# Autodesk Inventor assembly: 19182 DSNU-8-100-P-A---(0)
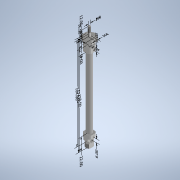
[picture p0: Inventor's stored thumbnail of the model, 180x180]
Saved by Autodesk Inventor 2021 (Build 250183000, 183)
## iProperties
Category: PARTsolutions
Company: FESTO
Created: 2026-04-16
Part Number: 19182 DSNU-8-100-P-A---(0)
Catalog Web Link: www.3dfindit.com
Description: DSNU-round cylinder
Vendor: FESTO
Document SubType Name: Assembly
Designer: psAdmin
Manufacturer: FESTO
Mass: 58.6 g
Surface Area: 124.069 cm^2
Volume: 11.6186 cm^3
Density: 5.04364 g/cm^3
Title: 19182 DSNU-8-100-P-A
Author: Cadenas PARTsolutions
Comments: round cylinder
PSOL_IDENT_0: {ATYP=ASSISTANT},{DATA=script=$CADENAS_DATA/23d-libs/festo/webfesto.vbb&M_FAMILY=DSNU&M_GROUP=01&M_P
PSOL_IDENT_1: ARTNO=19182&IDCODE1=DSNU-8-100-P-A&IDCODE2=&customer_number_cns=&MATES=1&LOD=HI&LOCKERP=0&SINGLEPART=
PSOL_IDENT_2: 1}
NB: 19182 DSNU-8-100-P-A---(0)
NN: DSNU
NT: round cylinder
NBSYN: $NB1.---($HUBST.)
LINA: 19182 DSNU-8-100-P-A
CATALOG: Festo
OFFICIAL_STANDARD_NUMBERS: ISO 6432
TNR: 19182
TYP: DSNU-8
KDM: 8
HUB: 100
HUBST: 0
DA: P
PE: A
KS: -
A1: 15
A2: 50
A3: 4
A4: 29
AB: 12
AM: 12
B: 12
BB: 3
BE: M12x1,25
BS: 3.4
B1: 24
B2: 0
B3: 0
B4: 0
B5: 14
B6: 6
B7: 0
CD: 4
D: 15
D1: 12
D2: 4
D3: 9.3
D4: 0
D5: 10.5
D6: 0
D7: 0
EE: M5
EW: 8
F: 18
FF: M3
F1: 0
H: 16
H1: 0
KK: M4
K1: -
K2: 0
KV: 19
KW: 6
KV2: 0
KW2: 0
L: 6
LH: 5
LK: 7.6
L1: 174
L2: 146
L3: 6
L4: 12
L5: 10
L6: 28
L7: 16
L8: 10
L9: 16
L13: 78
ST: 3.4
SW: 0
T: 0
WH: 16
X: 0
XC: 164
CNSMASSEXACT: 0.0586
GTIN: 4052568066949
REACH: Yes
REACHSVHC: No
REACHHAZSUBS: -
REACHSCIP: -
REACHVALDATE: -
SUPPLIER: FESTO
ARTICLENO: 19182 DSNU-8-100-P-A---(0)
BOMINFO: 19182 DSNU-8-100-P-A
CREATOR: CADENAS GmbH
## Documents named in this file (4)
- e:\temp\worker_COMMON_20\temp\tmp_2484_30_KxpFe\format_0\19182 DSNU-8-100-P-A---(0).iam
- e:\temp\worker_COMMON_20\temp\tmp_2484_30_KxpFe\format_0\19182 DSNU-8-100-P---(A----0-ZR).ipt
- e:\temp\worker_COMMON_20\temp\tmp_2484_30_KxpFe\format_0\DIN-439-B - M12x1_25(F).ipt
- e:\temp\worker_COMMON_20\temp\tmp_2484_30_KxpFe\format_0\19182 DSNU-8-100-P---(A---00--0-KS).ipt
## Components (3 placed, 3 different names)
1. 19182 DSNU-8-100-P---(A----0-ZR):1 — NUT_XY@1 <-> 2CYL_XY@2, NUT_Z@1 <-> 2CYL_Z@2, NUT_YZ@1 <-> 2CYL_YZ@2, ZR_XY@1 <-> KS_XY@3, ZR_Z@1 <-> KS_Z@3, ZR_YZ@1 <-> KS_YZ@3
2. DIN-439-B - M12x1_25(F):1 — NUT_XY@1 <-> 2CYL_XY@2, NUT_Z@1 <-> 2CYL_Z@2, NUT_YZ@1 <-> 2CYL_YZ@2
3. 19182 DSNU-8-100-P---(A---00--0-KS):1 — ZR_XY@1 <-> KS_XY@3, ZR_Z@1 <-> KS_Z@3, ZR_YZ@1 <-> KS_YZ@3
## Relationships (6: Mate 4, Angle 2)
- NUT_XY@1 <-> 2CYL_XY@2 [Mate] (-3 mm): 19182 DSNU-8-100-P---(A----0-ZR):1 ↔ DIN-439-B - M12x1_25(F):1
- NUT_Z@1 <-> 2CYL_Z@2 [Mate]: 19182 DSNU-8-100-P---(A----0-ZR):1 ↔ DIN-439-B - M12x1_25(F):1
- NUT_YZ@1 <-> 2CYL_YZ@2 [Angle] (0 deg): 19182 DSNU-8-100-P---(A----0-ZR):1 ↔ DIN-439-B - M12x1_25(F):1
- ZR_XY@1 <-> KS_XY@3 [Mate]: 19182 DSNU-8-100-P---(A----0-ZR):1 ↔ 19182 DSNU-8-100-P---(A---00--0-KS):1
- ZR_Z@1 <-> KS_Z@3 [Mate]: 19182 DSNU-8-100-P---(A----0-ZR):1 ↔ 19182 DSNU-8-100-P---(A---00--0-KS):1
- ZR_YZ@1 <-> KS_YZ@3 [Angle] (0 deg): 19182 DSNU-8-100-P---(A----0-ZR):1 ↔ 19182 DSNU-8-100-P---(A---00--0-KS):1
